# Autodesk Inventor assembly: AnetUpgrade
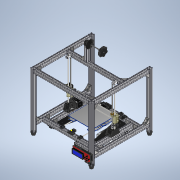
[picture p0: Inventor's stored thumbnail of the model, 180x180]
Saved by Autodesk Inventor 2020.2 (Build 242310000, 310)
## iProperties
Created: 2020-07-29
Part Number: AnetUpgrade
Document SubType Name: Assembly
Designer: JK
Author: JK
## Documents named in this file (14)
- C:\Users\JK\Documents\Inventor\Anet Upgrade\AnetUpgrade.iam
- C:\Users\JK\Documents\Inventor\Anet Upgrade\Frame.iam
- C:\Users\JK\Documents\Inventor\Anet Upgrade\xzrailassembly.iam
- C:\Users\JK\Documents\Inventor\Anet Upgrade\LCDassembly.iam
- C:\Users\JK\Documents\Inventor\Anet Upgrade\YIdlePulleyAssembly.iam
- C:\Users\JK\Documents\Inventor\Anet Upgrade\ButtonAssembly.iam
- C:\Users\JK\Documents\Inventor\Anet Upgrade\BedAssembly.iam
- C:\Users\JK\Documents\Inventor\Anet Upgrade\YMotorassembly.iam
- C:\Users\JK\Documents\Inventor\Anet Upgrade\Spoolholder.iam
- C:\Users\JK\Documents\Inventor\Anet Upgrade\BoardMount.iam
- C:\Users\JK\Documents\Inventor\Anet Upgrade\SocketAssembly.iam
- C:\Users\JK\Documents\Inventor\Anet Upgrade\ZEndStopAssembly.iam
- C:\Users\JK\Documents\Inventor\Anet Upgrade\PSUMount.iam
- C:\Users\JK\Documents\Inventor\Anet Upgrade\YEndstopAssembly.iam
## Components (13 placed, 13 different names)
1. Frame:1 [sub-assembly] — Angle:5, Mate:25, Flush:13, Flush:14, Mate:26, Flush:15, Mate:27, Flush:16, Flush:17, Mate:28, Flush:18, Flush:19, Flush:20, Mate:29, Flush:21, Flush:22, Mate:30, Flush:23, Mate:31, Mate:34, Flush:25, Flush:26, Flush:27, Mate:35, Flush:29, Flush:30, Mate:36, Mate:37, Mate:38, Flush:31
2. xzrailassembly:1 [sub-assembly] — Angle:5, Mate:36, Mate:37
3. LCDassembly:1 [sub-assembly] — Mate:25, Flush:13, Flush:14
4. YIdlePulleyAssembly:1 [sub-assembly] — Mate:26, Flush:15, Flush:20
5. ButtonAssembly:1 [sub-assembly] — Mate:27, Flush:16, Flush:17
6. BedAssembly:1 [sub-assembly] — Mate:28, Flush:18, Flush:19
7. YMotorassembly:1 [sub-assembly] — Mate:29, Flush:21, Flush:22
8. Spoolholder:1 [sub-assembly] — Mate:30, Flush:23, Mate:31
9. BoardMount:1 [sub-assembly] — Mate:34, Flush:25, Flush:28, Flush:29
10. SocketAssembly:1 [sub-assembly] — Flush:26, Flush:27
11. ZEndStopAssembly:1 [sub-assembly]
12. PSUMount:1 [sub-assembly] — Mate:35, Flush:28, Flush:30
13. YEndstopAssembly:1 [sub-assembly] — Mate:38, Flush:31
## Relationships (36: Flush 18, Mate 14, Angle 4)
- Angle:5 (0 deg): Frame:1 ↔ xzrailassembly:1
- Mate:25: Frame:1 ↔ LCDassembly:1
- Flush:13 (8.5 mm): Frame:1 ↔ LCDassembly:1
- Flush:14 (-11 mm): Frame:1 ↔ LCDassembly:1
- Mate:26: Frame:1 ↔ YIdlePulleyAssembly:1
- Flush:15: Frame:1 ↔ YIdlePulleyAssembly:1
- Mate:27: Frame:1 ↔ ButtonAssembly:1
- Flush:16: Frame:1 ↔ ButtonAssembly:1
- Flush:17 (-35 mm): Frame:1 ↔ ButtonAssembly:1
- Mate:28: Frame:1 ↔ BedAssembly:1
- Flush:18: Frame:1 ↔ BedAssembly:1
- Flush:19 (187.5 mm): Frame:1 ↔ BedAssembly:1
- Flush:20 (257 mm): Frame:1 ↔ YIdlePulleyAssembly:1
- Mate:29: Frame:1 ↔ YMotorassembly:1
- Flush:21: Frame:1 ↔ YMotorassembly:1
- Flush:22 (226 mm): Frame:1 ↔ YMotorassembly:1
- Mate:30: Frame:1 ↔ Spoolholder:1
- Flush:23: Frame:1 ↔ Spoolholder:1
- Mate:31: Frame:1 ↔ Spoolholder:1
- [Mate]: Frame:1 ↔ SocketAssembly:1
- [Angle] (0 deg): Frame:1 ↔ SocketAssembly:1
- [Mate]: xzrailassembly:1 ↔ ZEndStopAssembly:1
- Mate:34: Frame:1 ↔ BoardMount:1
- Flush:25 (1 mm): Frame:1 ↔ BoardMount:1
- Flush:26 (10 mm): Frame:1 ↔ SocketAssembly:1
- Flush:27 (50 mm): Frame:1 ↔ SocketAssembly:1
- [Angle] (0 deg): Frame:1 ↔ ZEndStopAssembly:1
- [Angle] (0 deg): xzrailassembly:1 ↔ ZEndStopAssembly:1
- Mate:35: Frame:1 ↔ PSUMount:1
- Flush:28: BoardMount:1 ↔ PSUMount:1
- Flush:29 (-4 mm): Frame:1 ↔ BoardMount:1
- Flush:30 (1 mm): Frame:1 ↔ PSUMount:1
- Mate:36: Frame:1 ↔ xzrailassembly:1
- Mate:37: Frame:1 ↔ xzrailassembly:1
- Mate:38: Frame:1 ↔ YEndstopAssembly:1
- Flush:31: Frame:1 ↔ YEndstopAssembly:1
